# Autodesk Inventor assembly: linear_cutting_endeffector-3
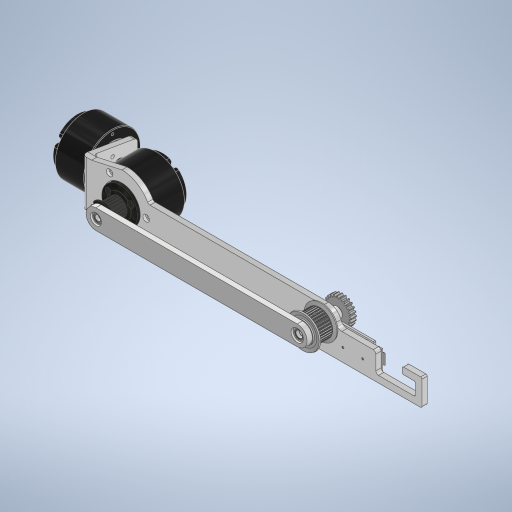
[picture p0: Inventor's stored thumbnail of the model, 512x512]
Saved by Autodesk Inventor 2024 (Build 280153000, 153)
## iProperties
Created: 2025-06-12
Part Number: linear_cutting_endeffector-3
Document SubType Name: Assembly
Designer: 1412z
Author: 1412z
## Documents named in this file (17)
- C:\Users\1412z\OneDrive\デスクトップ\rdclab\harvesting_robot\harvesting_endeffector\linear_cutting_endeffector\linear_cutting_endeffector-3.iam
- C:\Users\1412z\OneDrive\デスクトップ\rdclab\harvesting_robot\harvesting_endeffector\linear_cutting_endeffector\motor_holder\motor_holder-4.ipt
- C:\Users\1412z\OneDrive\デスクトップ\rdclab\harvesting_robot\harvesting_endeffector\linear_cutting_endeffector\misumi\SSE2B6L-100_Autodesk_Inventor_2023_20250607\AIS2023\SSE2B6-100_r.ipt
- C:\Users\1412z\OneDrive\デスクトップ\rdclab\harvesting_robot\harvesting_endeffector\linear_cutting_endeffector\misumi\screw\NBK_SNZSM26\SNZS-M2-6.ipt
- C:\Users\1412z\OneDrive\デスクトップ\rdclab\harvesting_robot\harvesting_endeffector\linear_cutting_endeffector\misumi\SSE2B6L-100_Autodesk_Inventor_2023_20250607\AIS2023\SSEB6_b.ipt
- C:\Users\1412z\OneDrive\デスクトップ\rdclab\harvesting_robot\harvesting_endeffector\linear_cutting_endeffector\misumi\LRGEAM0.8KA-80-K2-B50_Autodesk_Inventor_2024_20250607\LRGEAM0_8KA-80-K2-B50.ipt
- C:\Users\1412z\OneDrive\デスクトップ\rdclab\harvesting_robot\harvesting_endeffector\linear_cutting_endeffector\GIM3505-08\GIM3505-8_with-driver.ipt
- C:\Users\1412z\OneDrive\デスクトップ\rdclab\harvesting_robot\harvesting_endeffector\linear_cutting_endeffector\cutter\pen_type_cutter_realsize.ipt
- C:\Users\1412z\OneDrive\デスクトップ\rdclab\harvesting_robot\harvesting_endeffector\linear_cutting_endeffector\misumi\meviy\slider_plate.ipt
- C:\Users\1412z\OneDrive\デスクトップ\rdclab\harvesting_robot\harvesting_endeffector\linear_cutting_endeffector\misumi\C-FL675ZZ_Autodesk_Inventor_2024_20250608\C-FL675ZZ.ipt
- C:\Users\1412z\OneDrive\デスクトップ\rdclab\harvesting_robot\harvesting_endeffector\linear_cutting_endeffector\misumi\simring\simring_Φ5-Φ7.ipt
- C:\Users\1412z\OneDrive\デスクトップ\rdclab\harvesting_robot\harvesting_endeffector\linear_cutting_endeffector\misumi\HTPA32S2M100-A-P5_Autodesk_Inventor_2024_20250608\AIS2024\HTPA32S2M100-A-P5.iam
- C:\Users\1412z\OneDrive\デスクトップ\rdclab\harvesting_robot\harvesting_endeffector\linear_cutting_endeffector\misumi\CLBPS5-8-6.3_Autodesk_Inventor_2024_20250612\CLBPS5-8-6_3.ipt
- C:\Users\1412z\OneDrive\デスクトップ\rdclab\harvesting_robot\harvesting_endeffector\linear_cutting_endeffector\misumi\M0.8-24\Spur Gear (24 teeth).ipt
- C:\Users\1412z\OneDrive\デスクトップ\rdclab\harvesting_robot\harvesting_endeffector\linear_cutting_endeffector\misumi\HTPA22S2M100-A-V4-Z6-J3_Autodesk_Inventor_2024_20250304\HTPA22S2M100-A-V4-Z6-J3_0_a-3.ipt
- C:\Users\1412z\OneDrive\デスクトップ\rdclab\harvesting_robot\harvesting_endeffector\linear_cutting_endeffector\motor_holder\motor_holder_top-2.ipt
- C:\Users\1412z\OneDrive\デスクトップ\rdclab\harvesting_robot\harvesting_endeffector\linear_cutting_endeffector\misumi\SFL674ZZ_Autodesk_Inventor_2024_20250304\SFL674ZZ.ipt
## Components (27 placed, 16 different names)
1. motor_holder-4:1 — 回転:1, 回転:2, 回転:12, 回転:13, 回転:14, 回転:15, 回転:20, 回転:21
2. SSE2B6-100_r:1 — 回転:1, 回転:2, 回転:3, 回転:4, 回転:5, 回転:6, 回転:7, 回転:8, 回転:9, 円柱状:1, 円柱状:2
3. SNZS-M2-6:1 — 回転:3
4. SNZS-M2-6:2 — 回転:4
5. SNZS-M2-6:3 — 回転:5
6. SNZS-M2-6:4 — 回転:6
7. SNZS-M2-6:5 — 回転:7
8. SNZS-M2-6:6 — 回転:8
9. SNZS-M2-6:7 — 回転:9
10. SSEB6_b:1 — 円柱状:1, 回転:17
11. SSEB6_b:2 — 円柱状:2, 回転:16
12. GIM3505-8_with-driver:1 — 回転:12, 回転:13, 回転:27, 回転:28
13. GIM3505-8_with-driver:2 — 回転:14, 回転:15
14. pen_type_cutter_realsize:1
15. slider_plate:1 — 回転:16, 回転:17, 回転:18, 回転:19
16. LRGEAM0_8KA-80-K2-B50:1 — 回転:18, 回転:19
17. C-FL675ZZ:1 — 回転:20, 回転:23
18. C-FL675ZZ:2 — 回転:21, 回転:22
19. simring_Φ5-Φ7:1 — 回転:23, 回転:25
20. simring_Φ5-Φ7:2 — 回転:22, 回転:24
21. HTPA32S2M100-A-P5:1 [sub-assembly] — 回転:24, 回転:29
22. CLBPS5-8-6_3:1 — 回転:25, 回転:26
23. Spur Gear (24 teeth):1 — 回転:26
24. HTPA22S2M100-A-V4-Z6-J3_0_a-3:1 — 回転:27, 回転:28, 回転:30
25. motor_holder_top-2:1 — 回転:29, 回転:30, 回転:31, 回転:32
26. SFL674ZZ:1 — 回転:31
27. C-FL675ZZ:3 — 回転:32
## Relationships (32: RevoluteJoint 30, CylindricalJoint 2)
- 回転:1 [RevoluteJoint]: motor_holder-4:1 ↔ SSE2B6-100_r:1
- 回転:2 [RevoluteJoint]: motor_holder-4:1 ↔ SSE2B6-100_r:1
- 回転:3 [RevoluteJoint]: SSE2B6-100_r:1 ↔ SNZS-M2-6:1
- 回転:4 [RevoluteJoint]: SSE2B6-100_r:1 ↔ SNZS-M2-6:2
- 回転:5 [RevoluteJoint]: SSE2B6-100_r:1 ↔ SNZS-M2-6:3
- 回転:6 [RevoluteJoint]: SSE2B6-100_r:1 ↔ SNZS-M2-6:4
- 回転:7 [RevoluteJoint]: SSE2B6-100_r:1 ↔ SNZS-M2-6:5
- 回転:8 [RevoluteJoint]: SSE2B6-100_r:1 ↔ SNZS-M2-6:6
- 回転:9 [RevoluteJoint]: SSE2B6-100_r:1 ↔ SNZS-M2-6:7
- 円柱状:1 [CylindricalJoint]: SSE2B6-100_r:1 ↔ SSEB6_b:1
- 円柱状:2 [CylindricalJoint]: SSE2B6-100_r:1 ↔ SSEB6_b:2
- 回転:12 [RevoluteJoint]: motor_holder-4:1 ↔ GIM3505-8_with-driver:1
- 回転:13 [RevoluteJoint]: motor_holder-4:1 ↔ GIM3505-8_with-driver:1
- 回転:14 [RevoluteJoint]: motor_holder-4:1 ↔ GIM3505-8_with-driver:2
- 回転:15 [RevoluteJoint]: motor_holder-4:1 ↔ GIM3505-8_with-driver:2
- 回転:16 [RevoluteJoint]: SSEB6_b:2 ↔ slider_plate:1
- 回転:17 [RevoluteJoint]: SSEB6_b:1 ↔ slider_plate:1
- 回転:18 [RevoluteJoint]: slider_plate:1 ↔ LRGEAM0_8KA-80-K2-B50:1
- 回転:19 [RevoluteJoint]: slider_plate:1 ↔ LRGEAM0_8KA-80-K2-B50:1
- 回転:20 [RevoluteJoint]: motor_holder-4:1 ↔ C-FL675ZZ:1
- 回転:21 [RevoluteJoint]: motor_holder-4:1 ↔ C-FL675ZZ:2
- 回転:22 [RevoluteJoint]: C-FL675ZZ:2 ↔ simring_Φ5-Φ7:2
- 回転:23 [RevoluteJoint]: C-FL675ZZ:1 ↔ simring_Φ5-Φ7:1
- 回転:24 [RevoluteJoint]: simring_Φ5-Φ7:2 ↔ HTPA32S2M100-A-P5:1
- 回転:25 [RevoluteJoint]: simring_Φ5-Φ7:1 ↔ CLBPS5-8-6_3:1
- 回転:26 [RevoluteJoint]: CLBPS5-8-6_3:1 ↔ Spur Gear (24 teeth):1
- 回転:27 [RevoluteJoint]: GIM3505-8_with-driver:1 ↔ HTPA22S2M100-A-V4-Z6-J3_0_a-3:1
- 回転:28 [RevoluteJoint]: GIM3505-8_with-driver:1 ↔ HTPA22S2M100-A-V4-Z6-J3_0_a-3:1
- 回転:29 [RevoluteJoint]: HTPA32S2M100-A-P5:1 ↔ motor_holder_top-2:1
- 回転:30 [RevoluteJoint]: HTPA22S2M100-A-V4-Z6-J3_0_a-3:1 ↔ motor_holder_top-2:1
- 回転:31 [RevoluteJoint]: motor_holder_top-2:1 ↔ SFL674ZZ:1
- 回転:32 [RevoluteJoint]: motor_holder_top-2:1 ↔ C-FL675ZZ:3
